# Autodesk Inventor assembly: PX9200-29A_Vacuum_Wheel_Complete
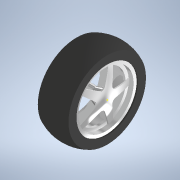
[picture p0: Inventor's stored thumbnail of the model, 180x180]
Saved by Autodesk Inventor 2022.3 (Build 263350000, 350)
## iProperties
Created: 2022-07-07
Part Number: PX9200-29A_Vacuum_Wheel_Complete
Document SubType Name: Assembly
Designer: luis_
Author: luis_
## Documents named in this file (3)
- D:\Luis\Desktop\ESPOL\9 semestre\Itinerario\PIEZAS\PX9200-29A_Vacuum_Wheel_Complete.iam
- D:\Luis\Desktop\ESPOL\9 semestre\Itinerario\PIEZAS\PX9200-29A_Wheel.ipt
- D:\Luis\Desktop\ESPOL\9 semestre\Itinerario\PIEZAS\PX9200-29B_Tire.ipt
## Components (2 placed, 2 different names)
1. PX9200-29A_Wheel:1 — Insert:1
2. PX9200-29B_Tire:1 — Insert:1
## Relationships (1: Insert 1)
- Insert:1: PX9200-29A_Wheel:1 ↔ PX9200-29B_Tire:1
